# Autodesk Inventor assembly: Wheel Module_MIR
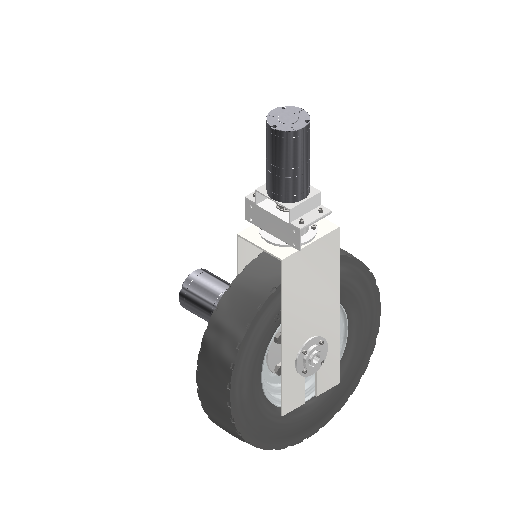
[picture p0: Inventor's stored thumbnail of the model, 512x512]
Saved by Autodesk Inventor 2022 (Build 260153000, 153)
## iProperties
Created: 2024-07-01
Part Number: Wheel Module_MIR
Document SubType Name: Assembly
Designer: LaptopJR
Author: LaptopJR
## Documents named in this file (24)
- C:\Users\LaptopJR\Documents\Ideation AI\EcoTerrabot\Chassis\CAD files\Wheel module\Wheel Module_MIR.iam
- C:\Users\LaptopJR\Documents\Ideation AI\EcoTerrabot\Chassis\CAD files\Wheel module\PA_402_4_G15_MIR.ipt
- C:\Users\LaptopJR\Documents\Ideation AI\EcoTerrabot\Chassis\CAD files\Wheel module\wheelFlange_MIR.ipt
- C:\Users\LaptopJR\Documents\Ideation AI\EcoTerrabot\Chassis\CAD files\Wheel module\wheelFlangeMotor_MIR.ipt
- C:\Users\LaptopJR\Documents\Ideation AI\EcoTerrabot\Chassis\CAD files\Wheel module\PL82Z-BL82.106-i3.65_MIR.ipt
- C:\Users\LaptopJR\Documents\Ideation AI\EcoTerrabot\Chassis\CAD files\Wheel module\Guide Pin_MIR.ipt
- C:\Users\LaptopJR\Documents\Ideation AI\EcoTerrabot\Chassis\CAD files\Wheel module\CShape_MIR.ipt
- C:\Users\LaptopJR\Documents\Ideation AI\EcoTerrabot\Chassis\CAD files\Wheel module\BearingHolder_MIR.ipt
- C:\Users\LaptopJR\Documents\Ideation AI\EcoTerrabot\Chassis\CAD files\Wheel module\Bearing 61806\skf_bearing_61806-2rs1_2_MIR.iam
- C:\Users\LaptopJR\Documents\Ideation AI\EcoTerrabot\Chassis\CAD files\Wheel module\MotorBracket_MIR.ipt
- C:\Users\LaptopJR\Documents\Inventor\Content Center Files\R2022\en-US\SS-ISO 4762\ISO 4762 - M6 x 16SS-ISO.ipt
- C:\Users\LaptopJR\Documents\Inventor\Content Center Files\R2022\en-US\DIN 934\DIN 934 - M6 x 1.ipt
- C:\Users\LaptopJR\Documents\Inventor\Content Center Files\R2022\en-US\SS-ISO 4762\ISO 4762 - M5 x 16SS-ISO.ipt
- C:\Users\LaptopJR\Documents\Inventor\Content Center Files\R2022\en-US\DIN 934\DIN 934 - M5 x 0.8.ipt
- C:\Users\LaptopJR\Documents\Inventor\Content Center Files\R2022\en-US\ANSI B18.2.1(3)\ANSI B18.2.1 - 9_16-12 UNC - 1.5(3).ipt
- C:\Users\LaptopJR\Documents\Inventor\Content Center Files\R2022\en-US\ANSI B18.2.2(09)\ANSI B18.2.2 - 9_16 - 12(2).ipt
- C:\Users\LaptopJR\Documents\Ideation AI\EcoTerrabot\Chassis\CAD files\Wheel module\wheelFlangeTopMotor_MIR.ipt
- C:\Users\LaptopJR\Documents\Ideation AI\EcoTerrabot\Chassis\CAD files\Wheel module\WheelHolder_MIR.ipt
- C:\Users\LaptopJR\Documents\Ideation AI\EcoTerrabot\Chassis\CAD files\Wheel module\WheelHolder_S1_MIR.ipt
- C:\Users\LaptopJR\Documents\Ideation AI\EcoTerrabot\Chassis\CAD files\Wheel module\WheelHolder_S2_MIR.ipt
- C:\Users\LaptopJR\Documents\Ideation AI\EcoTerrabot\Chassis\CAD files\Wheel module\bearing 6306 2rs1\skf_bearing_6306-2rs1_2_MIR.iam
- C:\Users\LaptopJR\Documents\Inventor\Content Center Files\R2022\en-US\ANSI AFBMA  8.1 KM\ANSI_AFBMA Std 8.1 - KM 6.ipt
- C:\Users\LaptopJR\Documents\Ideation AI\EcoTerrabot\Chassis\CAD files\Wheel module\bearing 51106\skf_bearing_51106_2_MIR.iam
- C:\Users\LaptopJR\Documents\Ideation AI\EcoTerrabot\Chassis\CAD files\Wheel module\TopMotorBracket_MIR.ipt
## Components (78 placed, 23 different names)
1. PA_402_4_G15_MIR:1
2. wheelFlange_MIR:1
3. wheelFlangeMotor_MIR:1
4. PL82Z-BL82.106-i3.65_MIR:1
5. Guide Pin_MIR:1
6. CShape_MIR:1
7. BearingHolder_MIR:1
8. BearingHolder_MIR:2
9. skf_bearing_61806-2rs1_2_MIR:1 [sub-assembly]
10. skf_bearing_61806-2rs1_2_MIR:2 [sub-assembly]
11. MotorBracket_MIR:1
12. SS ISO 4762 M6 x 16:1
13. SS ISO 4762 M6 x 16:2
14. SS ISO 4762 M6 x 16:3
15. SS ISO 4762 M6 x 16:4
16. wheelFlangeTopMotor_MIR:1
17. PL82Z-BL82.106-i3.65_MIR:2
18. WheelHolder_MIR:1
19. WheelHolder_S1_MIR:1
20. WheelHolder_S2_MIR:1
21. WheelHolder_S1_MIR:2
22. skf_bearing_6306-2rs1_2_MIR:1 [sub-assembly]
23. skf_bearing_6306-2rs1_2_MIR:2 [sub-assembly]
24. ANSI/AFBMA Std 8.1 KM (Metric) KM 6:1
25. skf_bearing_51106_2_MIR:1 [sub-assembly]
26. TopMotorBracket_MIR:1
27. SS ISO 4762 M6 x 16:7
28. SS ISO 4762 M6 x 16:8
29. SS ISO 4762 M6 x 16:9
30. SS ISO 4762 M6 x 16:10
31. SS ISO 4762 M6 x 16:5
32. DIN 934 - replaced by DIN EN 24032/28673/28674 M6:1
33. SS ISO 4762 M6 x 16:12
34. DIN 934 - replaced by DIN EN 24032/28673/28674 M6:4
35. SS ISO 4762 M6 x 16:13
36. DIN 934 - replaced by DIN EN 24032/28673/28674 M6:5
37. SS ISO 4762 M6 x 16:14
38. DIN 934 - replaced by DIN EN 24032/28673/28674 M6:6
39. SS ISO 4762 M6 x 16:11
40. DIN 934 - replaced by DIN EN 24032/28673/28674 M6:3
41. SS ISO 4762 M6 x 16:15
42. DIN 934 - replaced by DIN EN 24032/28673/28674 M6:7
43. SS ISO 4762 M6 x 16:16
44. DIN 934 - replaced by DIN EN 24032/28673/28674 M6:8
45. SS ISO 4762 M6 x 16:17
46. DIN 934 - replaced by DIN EN 24032/28673/28674 M6:9
47. Hex Cap Screw - Inch 9/16-12 UNC - 1.5:1
48. Hex Nut - Inch 9/16 - 12:1
49. Hex Cap Screw - Inch 9/16-12 UNC - 1.5:2
50. Hex Nut - Inch 9/16 - 12:2
51. Hex Cap Screw - Inch 9/16-12 UNC - 1.5:3
52. Hex Nut - Inch 9/16 - 12:3
53. Hex Cap Screw - Inch 9/16-12 UNC - 1.5:4
54. Hex Nut - Inch 9/16 - 12:4
55. SS ISO 4762 M5 x 16:2
56. DIN 934 - replaced by DIN EN 24032/28673/28674 M5:2
57. SS ISO 4762 M5 x 16:3
58. DIN 934 - replaced by DIN EN 24032/28673/28674 M5:3
59. SS ISO 4762 M5 x 16:4
60. DIN 934 - replaced by DIN EN 24032/28673/28674 M5:4
61. SS ISO 4762 M5 x 16:5
62. DIN 934 - replaced by DIN EN 24032/28673/28674 M5:5
63. SS ISO 4762 M5 x 16:1
64. DIN 934 - replaced by DIN EN 24032/28673/28674 M5:1
65. SS ISO 4762 M5 x 16:6
66. DIN 934 - replaced by DIN EN 24032/28673/28674 M5:6
67. SS ISO 4762 M5 x 16:7
68. DIN 934 - replaced by DIN EN 24032/28673/28674 M5:7
69. SS ISO 4762 M5 x 16:8
70. DIN 934 - replaced by DIN EN 24032/28673/28674 M5:8
71. SS ISO 4762 M6 x 16:6
72. DIN 934 - replaced by DIN EN 24032/28673/28674 M6:2
73. SS ISO 4762 M6 x 16:18
74. DIN 934 - replaced by DIN EN 24032/28673/28674 M6:10
75. SS ISO 4762 M6 x 16:19
76. DIN 934 - replaced by DIN EN 24032/28673/28674 M6:11
77. SS ISO 4762 M6 x 16:20
78. DIN 934 - replaced by DIN EN 24032/28673/28674 M6:12
## Component patterns: (4 elements, first: SS ISO 4762 M6 x 16:5 + DIN 934 - replaced by DIN EN 24032/28673/28674 M6:1), (4 elements, first: SS ISO 4762 M6 x 16:11 + DIN 934 - replaced by DIN EN 24032/28673/28674 M6:3), (4 elements, first: Hex Cap Screw - Inch 9/16-12 UNC - 1.5:1 + Hex Nut - Inch 9/16 - 12:1), (4 elements, first: SS ISO 4762 M5 x 16:2 + DIN 934 - replaced by DIN EN 24032/28673/28674 M5:2), (4 elements, first: SS ISO 4762 M5 x 16:1 + DIN 934 - replaced by DIN EN 24032/28673/28674 M5:1), (4 elements, first: SS ISO 4762 M6 x 16:6 + DIN 934 - replaced by DIN EN 24032/28673/28674 M6:2)
